# Autodesk Inventor assembly: Time
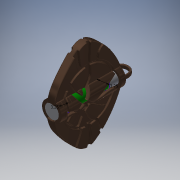
[picture p0: Inventor's stored thumbnail of the model, 180x180]
Saved by Autodesk Inventor 2019 (Build 230136000, 136)
## iProperties
Created: 2019-05-03
Part Number: Time
Document SubType Name: Assembly
Designer: Jorian Brusind
Author: Jorian Brusind
## Documents named in this file (4)
- C:\Users\Jorian Brusind\Documents\GitHub\PersonalProjects\Inventor Projects\Infinity\Time.iam
- C:\Users\Jorian Brusind\Documents\GitHub\PersonalProjects\Inventor Projects\Infinity\Green.ipt
- C:\Users\Jorian Brusind\Documents\GitHub\PersonalProjects\Inventor Projects\Infinity\Agamoto.ipt
- C:\Users\Jorian Brusind\Documents\GitHub\PersonalProjects\Inventor Projects\Infinity\EndCap.ipt
## Components (4 placed, 3 different names)
1. Green:1 — Mate:3, Mate:7
2. Agamoto:1 — Mate:3, Mate:4, Mate:5, Flush:1, Mate:6
3. EndCap:1 — Mate:4, Flush:1
4. EndCap:2 — Mate:5, Mate:6, Mate:7
## Relationships (6: Mate 5, Flush 1)
- Mate:3: Green:1 ↔ Agamoto:1
- Mate:4: Agamoto:1 ↔ EndCap:1
- Mate:5: Agamoto:1 ↔ EndCap:2
- Flush:1: Agamoto:1 ↔ EndCap:1
- Mate:6: Agamoto:1 ↔ EndCap:2
- Mate:7: Green:1 ↔ EndCap:2
